# Autodesk Inventor assembly: Sestava
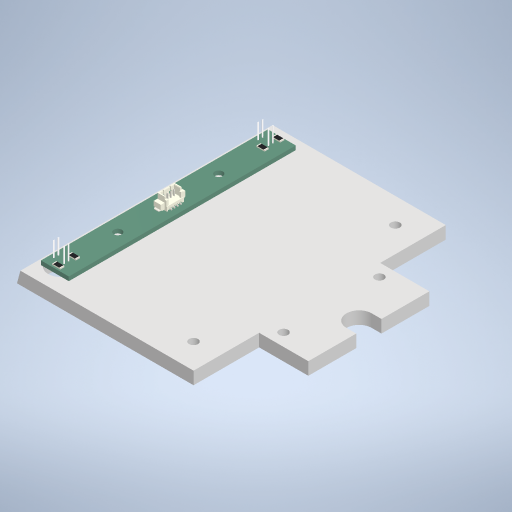
[picture p0: Inventor's stored thumbnail of the model, 512x512]
Saved by Autodesk Inventor 2024 (Build 280153000, 153)
## iProperties
Created: 2024-01-31
Part Number: Sestava
Document SubType Name: Assembly
Designer: Simak
Author: Simak
## Documents named in this file (3)
- C:\Users\Simak\OneDrive\Dokumenty\GitHub\RoboCop\- 3D -\_wip\Sestava.iam
- C:\Users\Simak\OneDrive\Dokumenty\GitHub\RoboCop\- 3D -\_wip\new_plech.ipt
- C:\Users\Simak\OneDrive\Dokumenty\GitHub\RoboCop\- 3D -\PCBs\QRE MiniBoards\QRE MiniBoards\QRE MiniBoards.iam
## Components (2 placed, 2 different names)
1. new_plech:1 — Proti sobě:1, Stejný směr:1, Stejný směr:2, Vložit:1
2. QRE MiniBoards:1 [sub-assembly] — Proti sobě:1, Stejný směr:1, Stejný směr:2, Vložit:1
## Relationships (4: Flush 2, Mate 1, Insert 1)
- Proti sobě:1 [Mate] (1 mm): new_plech:1 ↔ QRE MiniBoards:1
- Stejný směr:1 [Flush]: new_plech:1 ↔ QRE MiniBoards:1
- Stejný směr:2 [Flush] (5 mm): new_plech:1 ↔ QRE MiniBoards:1
- Vložit:1 [Insert]: new_plech:1 ↔ QRE MiniBoards:1
